# Autodesk Inventor assembly: uMule-Koło
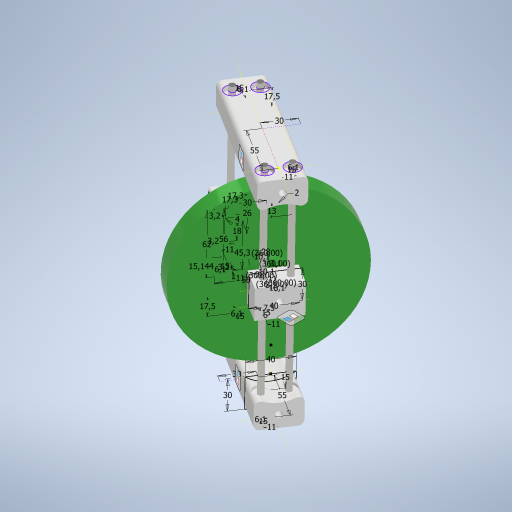
[picture p0: Inventor's stored thumbnail of the model, 512x512]
Saved by Autodesk Inventor 2024.3 (Build 283343000, 343)
## iProperties
Created: 2024-10-21
Part Number: uMule-Koło
Document SubType Name: Assembly
Designer: owozn
Author: owozn
## Documents named in this file (7)
- C:\Users\owozn\Documents\Nauka\Studia\mgr\Semestr_3\Magisterka\temp\uMule\mechanics\subsets\wheel\uMule-wheel_complete.iam
- C:\Users\owozn\Documents\Nauka\Studia\mgr\Semestr_3\Magisterka\temp\uMule\mechanics\subsets\wheel\uMule-wheel.ipt
- C:\Users\owozn\Documents\Nauka\Studia\mgr\Semestr_3\Magisterka\temp\uMule\mechanics\subsets\wheel\rx64H.ipt
- C:\Users\owozn\Documents\Nauka\Studia\mgr\Semestr_3\Magisterka\temp\uMule\mechanics\subsets\wheel\uMule-wheel_support.ipt
- C:\Users\owozn\Documents\Nauka\Studia\mgr\Semestr_3\Magisterka\temp\uMule\mechanics\subsets\wheel\uMule-wheel_limiter.ipt
- C:\Users\owozn\Documents\Nauka\Studia\mgr\Semestr_3\Magisterka\temp\uMule\mechanics\subsets\wheel\uMule-dx_top.ipt
- C:\Users\owozn\Documents\Nauka\Studia\mgr\Semestr_3\Magisterka\temp\uMule\mechanics\subsets\wheel\frame_rod.ipt
## Components (11 placed, 6 different names)
1. uMule-wheel:1 — Mate:1, Mate:2, Mate:3, Mate:4, Mate:7, Mate:21
2. uMule-wheel:2 — Mate:1, Mate:2, Mate:3, Mate:5
3. rx64H:1 — Mate:4, Mate:5, Flush:2, Mate:15, Mate:16
4. uMule-wheel_support:1 — Mate:7, Flush:3, Flush:4, Mate:19, Mate:21
5. uMule-wheel_limiter:1 — Flush:4, Flush:6, Mate:18, Mate:20, Mate:22, Mate:23, Mate:24, Flush:7, Flush:8, Flush:9
6. uMule-wheel_limiter:2 — Flush:3, Flush:5, Flush:6, Mate:17
7. uMule-dx_top:1 — Flush:2, Mate:15, Mate:16, Flush:5
8. frame_rod:1 — Mate:17, Mate:18, Mate:19, Mate:20
9. frame_rod:2 — Mate:22, Flush:7
10. frame_rod:3 — Mate:24, Flush:9
11. frame_rod:4 — Mate:23, Flush:8
## Relationships (24: Mate 16, Flush 8)
- Mate:1: uMule-wheel:1 ↔ uMule-wheel:2
- Mate:2: uMule-wheel:1 ↔ uMule-wheel:2
- Mate:3: uMule-wheel:1 ↔ uMule-wheel:2
- Mate:4: uMule-wheel:1 ↔ rx64H:1
- Mate:5: uMule-wheel:2 ↔ rx64H:1
- Mate:7 (4 mm): uMule-wheel:1 ↔ uMule-wheel_support:1
- Flush:2: rx64H:1 ↔ uMule-dx_top:1
- Mate:15: rx64H:1 ↔ uMule-dx_top:1
- Mate:16: rx64H:1 ↔ uMule-dx_top:1
- Flush:3 (100 mm): uMule-wheel_support:1 ↔ uMule-wheel_limiter:2
- Flush:4 (100 mm): uMule-wheel_support:1 ↔ uMule-wheel_limiter:1
- Flush:5 (5 mm): uMule-wheel_limiter:2 ↔ uMule-dx_top:1
- Flush:6: uMule-wheel_limiter:1 ↔ uMule-wheel_limiter:2
- Mate:17: uMule-wheel_limiter:2 ↔ frame_rod:1
- Mate:18: uMule-wheel_limiter:1 ↔ frame_rod:1
- Mate:19: uMule-wheel_support:1 ↔ frame_rod:1
- Mate:20 (5 mm): uMule-wheel_limiter:1 ↔ frame_rod:1
- Mate:21: uMule-wheel:1 ↔ uMule-wheel_support:1
- Mate:22: uMule-wheel_limiter:1 ↔ frame_rod:2
- Mate:23: uMule-wheel_limiter:1 ↔ frame_rod:4
- Mate:24: uMule-wheel_limiter:1 ↔ frame_rod:3
- Flush:7 (5 mm): uMule-wheel_limiter:1 ↔ frame_rod:2
- Flush:8 (-5 mm): uMule-wheel_limiter:1 ↔ frame_rod:4
- Flush:9 (5 mm): uMule-wheel_limiter:1 ↔ frame_rod:3
